# Autodesk Inventor assembly: StubAxle
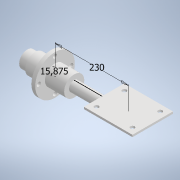
[picture p0: Inventor's stored thumbnail of the model, 180x180]
Saved by Autodesk Inventor 2020 (Build 240168000, 168)
## iProperties
Created: 2020-03-13
Part Number: StubAxle
Document SubType Name: Assembly
Designer: jgranlund
Author: jgranlund
## Documents named in this file (3)
- C:\Projects\SolarTracker\Inventor\TrackerFrame\Assembly\StubAxle.iam
- C:\Projects\SolarTracker\Inventor\TrackerFrame\Parts\Spindle.ipt
- C:\Projects\SolarTracker\Inventor\TrackerFrame\Parts\pilot.ipt
## Components (2 placed, 2 different names)
1. Spindle:1 — Cylindrical:1
2. pilot:1 — Cylindrical:1
## Relationships (1: CylindricalJoint 1)
- Cylindrical:1: Spindle:1 ↔ pilot:1
